# Autodesk Inventor assembly: Placed corner cabinet with step#2
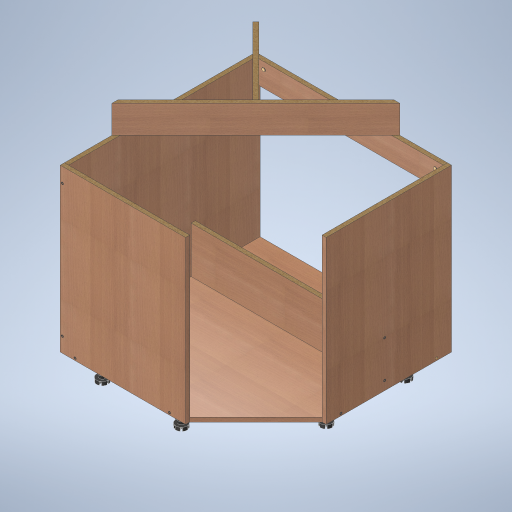
[picture p0: Inventor's stored thumbnail of the model, 512x512]
Saved by Autodesk Inventor 2024 (Build 280153000, 153)
## iProperties
Created: 2017-02-01
Part Number: Placed corner cabinet with step#2
Document SubType Name: Assembly
Designer: SvetlanaB
Author: SvetlanaB
## Documents named in this file (20)
- C:\W4INV 2024 Design\iBOX LIBRARY\Kitchen\Standing Cabinets\Corner cabinet with step#2\corner cabinet 2.iam
- C:\W4INV 2024 Design\iBOX LIBRARY\Kitchen\Standing Cabinets\Corner cabinet with step#2\Right panel.ipt
- C:\W4INV 2024 Design\iBOX LIBRARY\Kitchen\Standing Cabinets\Corner cabinet with step#2\Left panel.ipt
- C:\W4INV 2024 Design\iBOX LIBRARY\Kitchen\Standing Cabinets\Corner cabinet with step#2\Back panel.ipt
- C:\W4INV 2024 Design\iBOX LIBRARY\Kitchen\Standing Cabinets\Corner cabinet with step#2\Bottom panel.ipt
- C:\W4INV 2024 Design\iBOX LIBRARY\Kitchen\Standing Cabinets\Corner cabinet with step#2\Panel_1.ipt
- C:\W4INV 2024 Design\iBOX LIBRARY\Kitchen\Standing Cabinets\Corner cabinet with step#2\Panel_2.ipt
- C:\W4INV 2024 Design\iBOX LIBRARY\Kitchen\Standing Cabinets\Corner cabinet with step#2\Panel_3.ipt
- C:\W4INV 2024 Design\iBOX LIBRARY\Kitchen\Standing Cabinets\Corner cabinet with step#2\Panel_4.ipt
- C:\W4INV 2024 Design\_LIBRARY\Fixed joints\Minifix joint\MINIFIX D15 v2\Minifix D15 & Dowel L34 & Cap D15 PB T18 LH.ipt
- C:\W4INV 2024 Design\_LIBRARY\Supports and legs\Legs\ADJUSTABLE LEG\Adjustable leg  BT18 clip included.ipt
- C:\W4INV 2024 Design\_LIBRARY\Supports and legs\Legs\ADJUSTABLE LEG\Adjustable leg  BT18.ipt
- C:\W4INV 2024 Design\_LIBRARY\Fixed joints\Confirmat\CONFIRMAT\Confirmat L50 NB T18 PB T 18.ipt
- C:\W4INV 2024 Design\iBOX LIBRARY\Kitchen\Standing Cabinets\Corner cabinet with step#2\corner cabinet concept.ipt
- C:\W4INV 2024 Design\_LIBRARY\Fixed joints\Minifix joint\MINIFIX D15 v2\Minifix D15 & Dowel L34 & Cap D15 PB T18 RH.ipt
- C:\W4INV 2024 Design\_LIBRARY\Fixed joints\Confirmat\CONFIRMAT\Confirmat L50 & Cap D10 NB T18 PB T 18.ipt
- C:\W4INV 2024 Design\_LIBRARY\Fixed joints\Minifix joint\MINIFIX D15 v2\Minifix D15 & Dowel L34 & Cap D15 PB T18 BT.ipt
- C:\W4INV 2023 Design\LIBRARY\Fixed joints\Minifix joint\MINIFIX D15 v2.ipt
- C:\W4INV 2023 Design\LIBRARY\Fixed joints\Confirmat\CONFIRMAT.ipt
- C:\W4INV 2023 Design\LIBRARY\Supports and legs\Legs\ADJUSTABLE LEG.ipt
## Components (29 placed, 16 different names)
1. @Skeleton
2. Right panel:1 — Flush:3, Flush:4, Flush:16, Flush:18, Nestled Board Plane:1, Nestled Board Plane:2, Nestled Board Plane:12, Nestled Board Plane:14, Nestled Board Plane:4
3. Left panel:1 — Flush:2, Flush:6, Flush:19, Nestled Board Plane:5, Nestled Board Plane:6, Nestled Board Plane:8, Nestled Board Plane:10
4. Back panel:1 — Flush:5, Flush:7, Flush:20, Flush:24, Flush:25, Nestled Board Plane:7, Pillar Board Side Plane:8, Pillar Board Side Plane:9, Nestled Board Plane:11, Nestled Board Plane:13, Nestled Board Plane:15, Nestled Board Plane:3
5. Bottom panel:1 — Flush:17, Bottom board Plane:2, Bottom board Plane:4, Bottom board Plane:5, Bottom board Plane:1, Front (Angle) Plane:1, Bottom board Plane:3, Front (Angle) Plane:2, Pillar Board Side Plane:1, Pillar Board Side Plane:2, Pillar Board Side Plane:5, Pillar Board Side Plane:6, Pillar Board Side Plane:7, Pillar Board Side Plane:12
6. Panel_1:1 — Flush:1, Flush:23, Pillar Board Side Plane:10, Pillar Board Side Plane:11, Flush:39, Pillar Board Side Plane:13, Pillar Board Side Plane:14
7. Panel_2:1 — Flush:28, Pillar Board Side Plane :1, Pillar Board Side Plane :2
8. Panel_3:1 — Nestled Board Plane:9
9. Panel_4:1 — Flush:21, Pillar Board Side Plane :9
10. Adjustable leg  BT18:2 — Bottom board Plane:2, Axis Plane:10, Axis2 Plane:2
11. Adjustable leg  BT18:4 — Bottom board Plane:4, Axis Plane:12, Axis2 Plane:4
12. Adjustable leg  BT18:5 — Bottom board Plane:5, Axis Plane:13, Axis2 Plane:5
13. Adjustable leg  BT18 clip included:7 — Bottom board Plane:1, Axis Plane:9, Axis2 Plane:1, Front (Angle) Plane:1
14. Adjustable leg  BT18 clip included:8 — Bottom board Plane:3, Axis Plane:11, Axis2 Plane:3, Front (Angle) Plane:2
15. Minifix D15 & Dowel L34 & Cap D15 PB T18 BT:9 — Nestled Board Plane:9, Pillar Board Side Plane :9, Axis Plane:14
16. Confirmat L50 & Cap D10 NB T18 PB T 18:1 — Axis Plane:1, Nestled Board Plane:1, Pillar Board Side Plane:1
17. Confirmat L50 NB T18 PB T 18:2 — Axis Plane:2, Nestled Board Plane:2, Pillar Board Side Plane:2
18. Confirmat L50 NB T18 PB T 18:5 — Axis Plane:5, Nestled Board Plane:5, Pillar Board Side Plane:5
19. Confirmat L50 NB T18 PB T 18:6 — Axis Plane:6, Nestled Board Plane:6, Pillar Board Side Plane:6
20. Confirmat L50 NB T18 PB T 18:7 — Nestled Board Plane:7, Pillar Board Side Plane:7, Axis Plane:7
21. Confirmat L50 NB T18 PB T 18:8 — Axis Plane:8, Nestled Board Plane:8, Pillar Board Side Plane:8
22. Confirmat L50 NB T18 PB T 18:9 — Axis Plane:15, Nestled Board Plane:10, Pillar Board Side Plane:9
23. Confirmat L50 NB T18 PB T 18:10 — Nestled Board Plane:11, Pillar Board Side Plane:10, Axis Plane:16
24. Confirmat L50 NB T18 PB T 18:11 — Nestled Board Plane:12, Pillar Board Side Plane:11, Axis Plane:17
25. Confirmat L50 NB T18 PB T 18:12 — Nestled Board Plane:13, Pillar Board Side Plane:12, Axis Plane:18
26. Confirmat L50 NB T18 PB T 18:13 — Nestled Board Plane:14, Pillar Board Side Plane:13, Axis Plane:19
27. Confirmat L50 NB T18 PB T 18:14 — Nestled Board Plane:15, Pillar Board Side Plane:14, Axis Plane:20
28. Minifix D15 & Dowel L34 & Cap D15 PB T18 RH:10 — Nestled Board Plane:3, Pillar Board Side Plane :1, Axis Plane:3
29. Minifix D15 & Dowel L34 & Cap D15 PB T18 LH:11 — Nestled Board Plane:4, Pillar Board Side Plane :2, Axis Plane:4
## Relationships (80: Mate 45, Flush 33, Angle 2)
- Flush:1 (-20 mm): Panel_1:1
- Flush:2 (-70 mm): Left panel:1
- Flush:3 (-64 mm): Right panel:1
- Flush:4 (-64 mm): Right panel:1
- Flush:5 (-64 mm): Back panel:1
- Flush:6 (-64 mm): Left panel:1
- Flush:7 (-64 mm): Back panel:1
- Flush:16 (-100 mm): Right panel:1
- Flush:17 (-100 mm): Bottom panel:1
- Flush:18 (-100 mm): Right panel:1
- Flush:19 (-100 mm): Left panel:1
- Flush:20 (-100 mm): Back panel:1
- Bottom board Plane:2 [Mate]: Bottom panel:1 ↔ Adjustable leg  BT18:2
- Axis Plane:10 [Mate]: Adjustable leg  BT18:2
- Axis2 Plane:2 [Mate]: Adjustable leg  BT18:2
- Bottom board Plane:4 [Mate]: Bottom panel:1 ↔ Adjustable leg  BT18:4
- Axis Plane:12 [Mate]: Adjustable leg  BT18:4
- Axis2 Plane:4 [Mate]: Adjustable leg  BT18:4
- Bottom board Plane:5 [Mate]: Bottom panel:1 ↔ Adjustable leg  BT18:5
- Axis Plane:13 [Mate]: Adjustable leg  BT18:5
- Axis2 Plane:5 [Mate]: Adjustable leg  BT18:5
- Bottom board Plane:1 [Mate]: Bottom panel:1 ↔ Adjustable leg  BT18 clip included:7
- Axis Plane:9 [Mate]: Adjustable leg  BT18 clip included:7
- Axis2 Plane:1 [Mate]: Adjustable leg  BT18 clip included:7
- Front (Angle) Plane:1 [Angle] (0 deg): Bottom panel:1 ↔ Adjustable leg  BT18 clip included:7
- Bottom board Plane:3 [Mate]: Bottom panel:1 ↔ Adjustable leg  BT18 clip included:8
- Axis Plane:11 [Mate]: Adjustable leg  BT18 clip included:8
- Axis2 Plane:3 [Mate]: Adjustable leg  BT18 clip included:8
- Front (Angle) Plane:2 [Angle] (0 deg): Bottom panel:1 ↔ Adjustable leg  BT18 clip included:8
- Flush:21 (-60 mm): Panel_4:1
- Nestled Board Plane:9 [Mate]: Panel_3:1 ↔ Minifix D15 & Dowel L34 & Cap D15 PB T18 BT:9
- Pillar Board Side Plane :9 [Flush] (18 mm): Panel_4:1 ↔ Minifix D15 & Dowel L34 & Cap D15 PB T18 BT:9
- Axis Plane:14 [Mate]: Minifix D15 & Dowel L34 & Cap D15 PB T18 BT:9
- Flush:23 (-20 mm): Panel_1:1
- Flush:24 (-64 mm): Back panel:1
- Flush:25 (-64 mm): Back panel:1
- Axis Plane:1 [Mate]: Confirmat L50 & Cap D10 NB T18 PB T 18:1
- Nestled Board Plane:1 [Flush]: Right panel:1 ↔ Confirmat L50 & Cap D10 NB T18 PB T 18:1
- Pillar Board Side Plane:1 [Mate] (-9 mm): Bottom panel:1 ↔ Confirmat L50 & Cap D10 NB T18 PB T 18:1
- Axis Plane:2 [Mate]: Confirmat L50 NB T18 PB T 18:2
- Nestled Board Plane:2 [Flush]: Right panel:1 ↔ Confirmat L50 NB T18 PB T 18:2
- Pillar Board Side Plane:2 [Mate] (-9 mm): Bottom panel:1 ↔ Confirmat L50 NB T18 PB T 18:2
- Flush:28 (-30 mm): Panel_2:1
- Axis Plane:5 [Mate]: Confirmat L50 NB T18 PB T 18:5
- Nestled Board Plane:5 [Flush]: Left panel:1 ↔ Confirmat L50 NB T18 PB T 18:5
- Pillar Board Side Plane:5 [Mate] (-9 mm): Bottom panel:1 ↔ Confirmat L50 NB T18 PB T 18:5
- Axis Plane:6 [Mate]: Confirmat L50 NB T18 PB T 18:6
- Nestled Board Plane:6 [Flush]: Left panel:1 ↔ Confirmat L50 NB T18 PB T 18:6
- Pillar Board Side Plane:6 [Mate] (-9 mm): Bottom panel:1 ↔ Confirmat L50 NB T18 PB T 18:6
- Nestled Board Plane:7 [Flush]: Back panel:1 ↔ Confirmat L50 NB T18 PB T 18:7
- Pillar Board Side Plane:7 [Mate] (-9 mm): Bottom panel:1 ↔ Confirmat L50 NB T18 PB T 18:7
- Axis Plane:7 [Mate]: Confirmat L50 NB T18 PB T 18:7
- Axis Plane:8 [Mate]: Confirmat L50 NB T18 PB T 18:8
- Nestled Board Plane:8 [Flush]: Left panel:1 ↔ Confirmat L50 NB T18 PB T 18:8
- Pillar Board Side Plane:8 [Mate] (-9 mm): Back panel:1 ↔ Confirmat L50 NB T18 PB T 18:8
- Axis Plane:15 [Mate]: Confirmat L50 NB T18 PB T 18:9
- Nestled Board Plane:10 [Flush]: Left panel:1 ↔ Confirmat L50 NB T18 PB T 18:9
- Pillar Board Side Plane:9 [Mate] (-9 mm): Back panel:1 ↔ Confirmat L50 NB T18 PB T 18:9
- Nestled Board Plane:11 [Flush]: Back panel:1 ↔ Confirmat L50 NB T18 PB T 18:10
- Pillar Board Side Plane:10 [Mate] (-9 mm): Panel_1:1 ↔ Confirmat L50 NB T18 PB T 18:10
- Axis Plane:16 [Mate]: Confirmat L50 NB T18 PB T 18:10
- Nestled Board Plane:12 [Flush]: Right panel:1 ↔ Confirmat L50 NB T18 PB T 18:11
- Pillar Board Side Plane:11 [Mate] (-9 mm): Panel_1:1 ↔ Confirmat L50 NB T18 PB T 18:11
- Axis Plane:17 [Mate]: Confirmat L50 NB T18 PB T 18:11
- Nestled Board Plane:13 [Flush]: Back panel:1 ↔ Confirmat L50 NB T18 PB T 18:12
- Pillar Board Side Plane:12 [Mate] (-9 mm): Bottom panel:1 ↔ Confirmat L50 NB T18 PB T 18:12
- Axis Plane:18 [Mate]: Confirmat L50 NB T18 PB T 18:12
- Flush:39 (-180 mm): Panel_1:1
- Nestled Board Plane:14 [Flush]: Right panel:1 ↔ Confirmat L50 NB T18 PB T 18:13
- Pillar Board Side Plane:13 [Mate] (-9 mm): Panel_1:1 ↔ Confirmat L50 NB T18 PB T 18:13
- Axis Plane:19 [Mate]: Confirmat L50 NB T18 PB T 18:13
- Nestled Board Plane:15 [Flush]: Back panel:1 ↔ Confirmat L50 NB T18 PB T 18:14
- Pillar Board Side Plane:14 [Mate] (-9 mm): Panel_1:1 ↔ Confirmat L50 NB T18 PB T 18:14
- Axis Plane:20 [Mate]: Confirmat L50 NB T18 PB T 18:14
- Nestled Board Plane:3 [Mate]: Back panel:1 ↔ Minifix D15 & Dowel L34 & Cap D15 PB T18 RH:10
- Pillar Board Side Plane :1 [Flush] (18 mm): Panel_2:1 ↔ Minifix D15 & Dowel L34 & Cap D15 PB T18 RH:10
- Axis Plane:3 [Mate]: Minifix D15 & Dowel L34 & Cap D15 PB T18 RH:10
- Nestled Board Plane:4 [Mate]: Right panel:1 ↔ Minifix D15 & Dowel L34 & Cap D15 PB T18 LH:11
- Pillar Board Side Plane :2 [Flush] (18 mm): Panel_2:1 ↔ Minifix D15 & Dowel L34 & Cap D15 PB T18 LH:11
- Axis Plane:4 [Mate]: Minifix D15 & Dowel L34 & Cap D15 PB T18 LH:11
## Named parameters: Panel_thickness = 18 mm, Right_Attachment_Width = 560 mm, Space_For_Elevation = 440 mm, LeftAttachmentWidth = 560 mm, DoorSpace = 379.00923 mm, Elevation_Heigth = 120 mm
